# Autodesk Inventor assembly: body
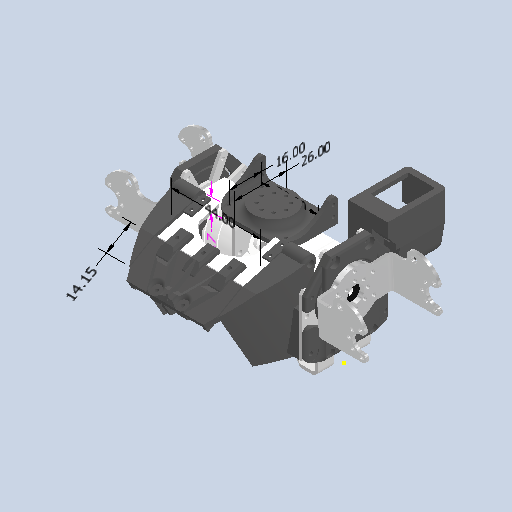
[picture p0: Inventor's stored thumbnail of the model, 512x512]
Saved by Autodesk Inventor 2024.1 (Build 281209000, 209)
## iProperties
Created: 2024-10-10
Part Number: body
Document SubType Name: Assembly
Designer: hibik
Author: hibik
## Documents named in this file (13)
- C:\Users\hibik\Documents\Robomech\HR\Eglantyne\hard\upper_body\upperbody.iam
- C:\Users\hibik\Documents\Robomech\HR\Eglantyne\hard\upper_body\body.ipt
- C:\Users\hibik\Documents\Robomech\HR\Eglantyne\hard\needed_model\KRS3300モータ.ipt
- C:\Users\hibik\Documents\Robomech\HR\Eglantyne\hard\needed_model\KRS3300サーボホーン.ipt
- C:\Users\hibik\Documents\Robomech\HR\Eglantyne\hard\upper_body\sholder.iam
- C:\Users\hibik\Documents\Robomech\HR\Eglantyne\hard\upper_body\chest\chest_right.iam
- C:\Users\hibik\Documents\Robomech\HR\Eglantyne\hard\upper_body\joit_cover_arm_under.ipt
- C:\Users\hibik\Documents\Robomech\HR\Eglantyne\hard\upper_body\joit_cover_arm_upper.ipt
- C:\Users\hibik\Documents\Robomech\HR\Eglantyne\hard\upper_body\neck_joint.ipt
- C:\Users\hibik\Documents\Robomech\HR\Eglantyne\hard\upper_body\chest\chest_base_left.ipt
- C:\Users\hibik\Documents\Robomech\HR\Eglantyne\hard\upper_body\neck.ipt
- C:\Users\hibik\Documents\Robomech\HR\Eglantyne\hard\upper_body\chest\chest_cover.iam
- C:\Users\hibik\Documents\Robomech\HR\Eglantyne\hard\upper_body\switch_setter.ipt
## Components (18 placed, 12 different names)
1. KRS3300モータ:1 — 挿入:4, 挿入:8, 角度:2, 挿入:12, 角度:4
2. KRS3300モータ:2 — 挿入:3, 挿入:7, 角度:1, 挿入:13, 挿入:14
3. KRS3300サーボホーン:1 — 挿入:3, 挿入:5
4. KRS3300サーボホーン:2 — 挿入:4, 挿入:6
5. sholder:1 [sub-assembly] — 挿入:5
6. sholder:2 [sub-assembly] — 挿入:6
7. chest_right:1 [sub-assembly] — 挿入:9, 挿入:10, 挿入:23, フラッシュ:1
8. joit_cover_arm_under:1 — 挿入:11, 角度:3
9. body:1 — 挿入:7, 角度:1, 挿入:8, 角度:2, 挿入:9, 挿入:10, 挿入:11, 角度:3, 挿入:15, 挿入:16, 挿入:17, 挿入:18, 挿入:19, 挿入:20, メイト:1, フラッシュ:2
10. joit_cover_arm_upper:1
11. neck_joint:1 — 挿入:12, 角度:4
12. neck_joint:2 — 挿入:13, 挿入:14, 挿入:21, 挿入:22
13. joit_cover_arm_under:2 — 挿入:16, 挿入:17
14. joit_cover_arm_upper:2 — 挿入:15, 挿入:18
15. chest_base_left:1 — 挿入:19, 挿入:20
16. neck:1 — 挿入:21, 挿入:22
17. chest_cover:1 [sub-assembly] — 挿入:23, フラッシュ:1
18. switch_setter:1 — メイト:1, フラッシュ:2
## Relationships (28: Insert 21, Angle 4, Flush 2, Mate 1)
- 挿入:3 [Insert]: KRS3300モータ:2 ↔ KRS3300サーボホーン:1
- 挿入:4 [Insert]: KRS3300モータ:1 ↔ KRS3300サーボホーン:2
- 挿入:5 [Insert]: KRS3300サーボホーン:1 ↔ sholder:1
- 挿入:6 [Insert]: KRS3300サーボホーン:2 ↔ sholder:2
- 挿入:7 [Insert]: KRS3300モータ:2 ↔ body:1
- 角度:1 [Angle] (180 deg): KRS3300モータ:2 ↔ body:1
- 挿入:8 [Insert]: KRS3300モータ:1 ↔ body:1
- 角度:2 [Angle] (180 deg): KRS3300モータ:1 ↔ body:1
- 挿入:9 [Insert]: chest_right:1 ↔ body:1
- 挿入:10 [Insert]: chest_right:1 ↔ body:1
- 挿入:11 [Insert]: joit_cover_arm_under:1 ↔ body:1
- 角度:3 [Angle] (180 deg): joit_cover_arm_under:1 ↔ body:1
- 挿入:12 [Insert]: KRS3300モータ:1 ↔ neck_joint:1
- 角度:4 [Angle] (0 deg): KRS3300モータ:1 ↔ neck_joint:1
- 挿入:13 [Insert]: KRS3300モータ:2 ↔ neck_joint:2
- 挿入:14 [Insert]: KRS3300モータ:2 ↔ neck_joint:2
- 挿入:15 [Insert]: body:1 ↔ joit_cover_arm_upper:2
- 挿入:16 [Insert]: body:1 ↔ joit_cover_arm_under:2
- 挿入:17 [Insert]: body:1 ↔ joit_cover_arm_under:2
- 挿入:18 [Insert]: body:1 ↔ joit_cover_arm_upper:2
- 挿入:19 [Insert]: body:1 ↔ chest_base_left:1
- 挿入:20 [Insert]: body:1 ↔ chest_base_left:1
- 挿入:21 [Insert]: neck_joint:2 ↔ neck:1
- 挿入:22 [Insert]: neck_joint:2 ↔ neck:1
- 挿入:23 [Insert] (0.5 mm): chest_right:1 ↔ chest_cover:1
- フラッシュ:1 [Flush]: chest_right:1 ↔ chest_cover:1
- メイト:1 [Mate]: body:1 ↔ switch_setter:1
- フラッシュ:2 [Flush]: body:1 ↔ switch_setter:1
